# Autodesk Inventor assembly: encoder-asm
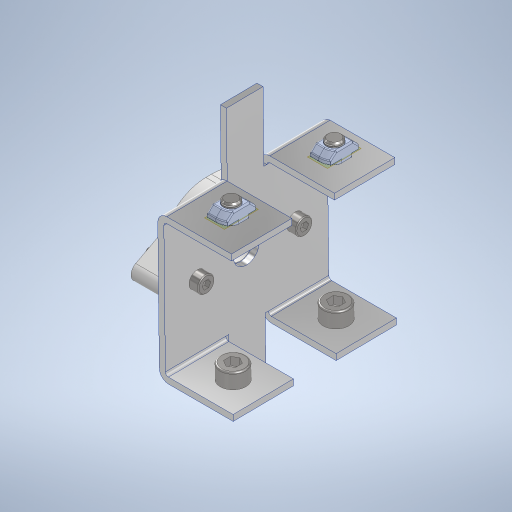
[picture p0: Inventor's stored thumbnail of the model, 512x512]
Saved by Autodesk Inventor 2024 (Build 280153000, 153)
## iProperties
Created: 2026-01-01
Part Number: encoder-asm
Document SubType Name: Assembly
Designer: schar
Author: schar
## Documents named in this file (4)
- C:\Users\schar\Desktop\projectBlueprint\AMSTS\hardware\encoder-asm.iam
- C:\Users\schar\Desktop\projectBlueprint\AMSTS\hardware\4x2020_encoder.iam
- C:\Users\schar\Desktop\projectBlueprint\AMSTS\hardware\tnut_m5_2020.ipt
- C:\Users\schar\Documents\Inventor\Content Center Files\R2024\en-US\ISO 4762(1)\DIN EN ISO 4762 - M5 x 8.ipt
## Components (9 placed, 3 different names)
1. 4x2020_encoder:1 [sub-assembly] — Rigid:1, Rigid:2, Rigid:3, Rigid:4, Mate:1, Mate:2, Mate:3, Mate:4
2. tnut_m5_2020:1 — Rigid:2, Mate:5
3. tnut_m5_2020:2 — Rigid:1, Mate:6
4. tnut_m5_2020:3 — Rigid:4, Mate:8
5. tnut_m5_2020:4 — Rigid:3, Mate:7
6. DIN EN ISO 4762 M5 x 8:1 — Mate:4, Mate:5
7. DIN EN ISO 4762 M5 x 8:2 — Mate:3, Mate:6
8. DIN EN ISO 4762 M5 x 8:3 — Mate:2, Mate:8
9. DIN EN ISO 4762 M5 x 8:4 — Mate:1, Mate:7
## Relationships (12: Mate 8, WeldJoint 4)
- Rigid:1 [WeldJoint] (-0.159 mm): 4x2020_encoder:1 ↔ tnut_m5_2020:2
- Rigid:2 [WeldJoint] (-0.159 mm): 4x2020_encoder:1 ↔ tnut_m5_2020:1
- Rigid:3 [WeldJoint] (-0.159 mm): 4x2020_encoder:1 ↔ tnut_m5_2020:4
- Rigid:4 [WeldJoint] (-0.159 mm): 4x2020_encoder:1 ↔ tnut_m5_2020:3
- Mate:1: 4x2020_encoder:1 ↔ DIN EN ISO 4762 M5 x 8:4
- Mate:2: 4x2020_encoder:1 ↔ DIN EN ISO 4762 M5 x 8:3
- Mate:3: 4x2020_encoder:1 ↔ DIN EN ISO 4762 M5 x 8:2
- Mate:4: 4x2020_encoder:1 ↔ DIN EN ISO 4762 M5 x 8:1
- Mate:5: tnut_m5_2020:1 ↔ DIN EN ISO 4762 M5 x 8:1
- Mate:6: tnut_m5_2020:2 ↔ DIN EN ISO 4762 M5 x 8:2
- Mate:7: tnut_m5_2020:4 ↔ DIN EN ISO 4762 M5 x 8:4
- Mate:8: tnut_m5_2020:3 ↔ DIN EN ISO 4762 M5 x 8:3
